# Autodesk Inventor assembly: motor_channel_mirrored
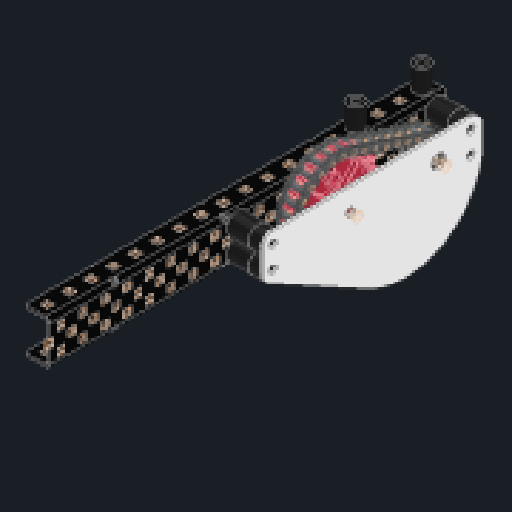
[picture p0: Inventor's stored thumbnail of the model, 512x512]
Saved by Autodesk Inventor 2024 (Build 280153000, 153)
## iProperties
Created: 2024-02-22
Part Number: motor_channel_mirrored
Document SubType Name: Assembly
Designer: Averey Ku
Author: Averey Ku
## Documents named in this file (16)
- D:\vex_robotics\hardware\cad\smolbot\intake\mirrored_parts\motor_channel_mirrored.iam
- D:\vex_robotics\hardware\cad\smolbot\intake\mirrored_parts\Alu C 1x2x1x18_mirrored.ipt
- D:\vex_robotics\hardware\cad\smolbot\intake\mirrored_parts\HS Bearing Flat_mirrored.ipt
- D:\vex_robotics\hardware\cad\smolbot\intake\mirrored_parts\intake_sled_mirrored.ipt
- D:\vex_robotics\hardware\cad\VEX-CAD-Inventor-1.41\Motion\Spacers\Spacer Nylon .375 OD\NSpacer .375 OD x .500.ipt
- D:\vex_robotics\hardware\cad\VEX-CAD-Inventor-1.41\Motion\Spacers\Spacer Nylon .375 OD.ipt
- D:\vex_robotics\hardware\cad\VEX-CAD-Inventor-1.41\Structure\Standoff\Standoff .875.ipt
- D:\vex_robotics\hardware\cad\VEX-CAD-Inventor-1.41\Structure\Standoff.ipt
- D:\vex_robotics\hardware\cad\VEX-CAD-Inventor-1.41\Motion\Sprockets\6P Sprocket\6P 8T Sprocket, No Insert.iam
- D:\vex_robotics\hardware\cad\VEX-CAD-Inventor-1.41\Motion\Sprockets\6P Sprocket.iam
- D:\vex_robotics\hardware\cad\VEX-CAD-Inventor-1.41\Motion\Sprockets\6P Sprocket\6P 24T Sprocket, No Insert.iam
- D:\vex_robotics\hardware\cad\smolbot\intake\chain.ipt
- D:\vex_robotics\hardware\cad\VEX-CAD-Inventor-1.41\Motion\Spacers\Spacer Nylon .500 OD\NSpacer Black .500 OD x .250.ipt
- D:\vex_robotics\hardware\cad\VEX-CAD-Inventor-1.41\Motion\Spacers\Spacer Nylon .500 OD.ipt
- D:\vex_robotics\hardware\cad\VEX-CAD-Inventor-1.41\Motion\Spacers\Spacer Nylon .500 OD\NSpacer Black .500 OD x .500.ipt
- D:\vex_robotics\hardware\cad\VEX-CAD-Inventor-1.41\Electronics\V5 Motor (5.5W).ipt
## Components (19 placed, 11 different names)
1. Alu C 1x2x1x18_mirrored:1 — Mate:1, Insert:5, Insert:13, Insert:14, Insert:16, Insert:17, Mate:2, Insert:21, Insert:23, Insert:27, Insert:28, Insert:29, Insert:30, Insert:31, Mate:5
2. HS Bearing Flat_mirrored:1 — Mate:1, Insert:5
3. intake_sled_mirrored:1 — Mate:2, Insert:24, Mate:4
4. NSpacer .375 OD x .500:1 — Insert:13
5. NSpacer .375 OD x .500:2 — Insert:14
6. Standoff .875:1 — Insert:16
7. Standoff .875:2 — Insert:17
8. 6P 8T Sprocket, No Insert:1 [sub-assembly] — Insert:30
9. 6P 24T Sprocket, No Insert:2 [sub-assembly] — Insert:29
10. chain:1
11. NSpacer Black .500 OD x .250:1 — Insert:24
12. NSpacer Black .500 OD x .500:2 — Insert:21
13. NSpacer Black .500 OD x .250:3 — Mate:4
14. NSpacer Black .500 OD x .500:4 — Insert:23
15. NSpacer Black .500 OD x .250:5
16. NSpacer Black .500 OD x .500:6 — Insert:27
17. NSpacer Black .500 OD x .250:7
18. NSpacer Black .500 OD x .500:8 — Insert:28
19. V5 Motor (5.5W):1 — Insert:31, Mate:5
## Relationships (23: Insert 18, Mate 5)
- Mate:1: Alu C 1x2x1x18_mirrored:1 ↔ HS Bearing Flat_mirrored:1
- Insert:5: Alu C 1x2x1x18_mirrored:1 ↔ HS Bearing Flat_mirrored:1
- Insert:13: Alu C 1x2x1x18_mirrored:1 ↔ NSpacer .375 OD x .500:1
- Insert:14: Alu C 1x2x1x18_mirrored:1 ↔ NSpacer .375 OD x .500:2
- Insert:16: Alu C 1x2x1x18_mirrored:1 ↔ Standoff .875:1
- Insert:17: Alu C 1x2x1x18_mirrored:1 ↔ Standoff .875:2
- Mate:2: Alu C 1x2x1x18_mirrored:1 ↔ intake_sled_mirrored:1
- [Insert] (6.35 mm): 6P 24T Sprocket, No Insert:2 ↔ chain:1
- [Mate]: 6P 8T Sprocket, No Insert:1 ↔ chain:1
- [Insert]: NSpacer Black .500 OD x .250:1 ↔ NSpacer Black .500 OD x .500:2
- Insert:21: Alu C 1x2x1x18_mirrored:1 ↔ NSpacer Black .500 OD x .500:2
- [Insert]: NSpacer Black .500 OD x .250:3 ↔ NSpacer Black .500 OD x .500:4
- Insert:23: Alu C 1x2x1x18_mirrored:1 ↔ NSpacer Black .500 OD x .500:4
- Insert:24: intake_sled_mirrored:1 ↔ NSpacer Black .500 OD x .250:1
- Mate:4: intake_sled_mirrored:1 ↔ NSpacer Black .500 OD x .250:3
- [Insert]: NSpacer Black .500 OD x .250:5 ↔ NSpacer Black .500 OD x .500:6
- [Insert]: NSpacer Black .500 OD x .250:7 ↔ NSpacer Black .500 OD x .500:8
- Insert:27: Alu C 1x2x1x18_mirrored:1 ↔ NSpacer Black .500 OD x .500:6
- Insert:28: Alu C 1x2x1x18_mirrored:1 ↔ NSpacer Black .500 OD x .500:8
- Insert:29 (3.175 mm): Alu C 1x2x1x18_mirrored:1 ↔ 6P 24T Sprocket, No Insert:2
- Insert:30 (3.175 mm): Alu C 1x2x1x18_mirrored:1 ↔ 6P 8T Sprocket, No Insert:1
- Insert:31: Alu C 1x2x1x18_mirrored:1 ↔ V5 Motor (5.5W):1
- Mate:5: Alu C 1x2x1x18_mirrored:1 ↔ V5 Motor (5.5W):1
## Named parameters: d24_d22 = 6.35 mm, d25_d23 = 0 mm, d28_d2 = 0 mm, d32_d2 = 0 mm, d33_d2 = 0 mm
